# Autodesk Inventor assembly: steelSlides350mm3.0
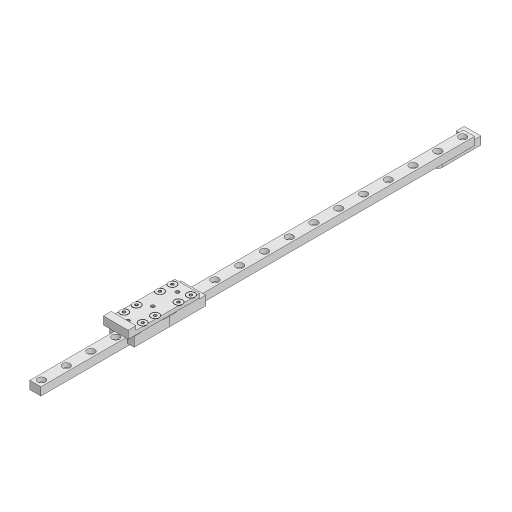
[picture p0: Inventor's stored thumbnail of the model, 512x512]
Saved by Autodesk Inventor 2023 (Build 270158000, 158)
## iProperties
Created: 2022-09-16
Part Number: steelSlides350mm3.0
Document SubType Name: Assembly
Designer: deli
Author: deli
## Documents named in this file (7)
- C:\Users\deli\OneDrive - Eastside Preparatory School\FTC\8103-power-play\CAD\steelSlides350mm3.0.iam
- C:\Users\deli\OneDrive - Eastside Preparatory School\FTC\8103-power-play\CAD\Rail.ipt
- C:\Users\deli\OneDrive - Eastside Preparatory School\FTC\8103-power-play\CAD\Carrige.ipt
- C:\Users\deli\OneDrive - Eastside Preparatory School\FTC\8103-power-play\CAD\Carrige Attatchment.ipt
- C:\Users\deli\OneDrive - Eastside Preparatory School\FTC\8103-power-play\CAD\FTC-parts\Mcmaster Carr\91294A126_Black-Oxide Alloy Steel Hex Drive Flat Head Screw.ipt
- C:\Users\deli\OneDrive - Eastside Preparatory School\FTC\8103-power-play\CAD\mgn9 350mm.ipt
- C:\Users\deli\OneDrive - Eastside Preparatory School\FTC\8103-power-play\CAD\mgn9SlideBearingHolder.ipt
## Components (14 placed, 6 different names)
1. Carrige:3 — Flush:1, Flush:2, Mate:1, Mate:9, Mate:10
2. Carrige:4 — Flush:1, Flush:2, Mate:1, Mate:4, Mate:22, Mate:23
3. Carrige Attatchment:1 — Mate:4, Mate:9, Mate:10, Mate:11, Mate:12, Mate:13, Mate:14, Mate:15, Mate:16, Mate:17, Mate:18, Mate:19, Mate:20, Mate:21, Flush:3, Flush:4, Flush:5, Flush:6, Flush:7, Flush:8, Flush:9, Flush:10
4. Rail:2 — Mate:11, Mate:12, Mate:13
5. 91294A126_Black-Oxide Alloy Steel Hex Drive Flat Head Screw:1 — Mate:20, Flush:8
6. 91294A126_Black-Oxide Alloy Steel Hex Drive Flat Head Screw:2 — Mate:21, Flush:10
7. 91294A126_Black-Oxide Alloy Steel Hex Drive Flat Head Screw:3 — Mate:16, Flush:4
8. 91294A126_Black-Oxide Alloy Steel Hex Drive Flat Head Screw:4 — Mate:15, Flush:3
9. 91294A126_Black-Oxide Alloy Steel Hex Drive Flat Head Screw:5 — Mate:17, Flush:7
10. 91294A126_Black-Oxide Alloy Steel Hex Drive Flat Head Screw:6 — Mate:18, Flush:6
11. 91294A126_Black-Oxide Alloy Steel Hex Drive Flat Head Screw:7 — Mate:19, Flush:9
12. 91294A126_Black-Oxide Alloy Steel Hex Drive Flat Head Screw:8 — Mate:14, Flush:5
13. mgn9 350mm:1 — Mate:22, Mate:23, Mate:24, Mate:25, Mate:26
14. mgn9SlideBearingHolder:1 — Mate:24, Mate:25, Mate:26
## Relationships (30: Mate 20, Flush 10)
- Flush:1: Carrige:3 ↔ Carrige:4
- Flush:2: Carrige:3 ↔ Carrige:4
- Mate:1: Carrige:3 ↔ Carrige:4
- Mate:4: Carrige:4 ↔ Carrige Attatchment:1
- Mate:9: Carrige:3 ↔ Carrige Attatchment:1
- Mate:10: Carrige:3 ↔ Carrige Attatchment:1
- Mate:11: Carrige Attatchment:1 ↔ Rail:2
- Mate:12: Carrige Attatchment:1 ↔ Rail:2
- Mate:13: Carrige Attatchment:1 ↔ Rail:2
- Mate:14: Carrige Attatchment:1 ↔ 91294A126_Black-Oxide Alloy Steel Hex Drive Flat Head Screw:8
- Mate:15: Carrige Attatchment:1 ↔ 91294A126_Black-Oxide Alloy Steel Hex Drive Flat Head Screw:4
- Mate:16: Carrige Attatchment:1 ↔ 91294A126_Black-Oxide Alloy Steel Hex Drive Flat Head Screw:3
- Mate:17: Carrige Attatchment:1 ↔ 91294A126_Black-Oxide Alloy Steel Hex Drive Flat Head Screw:5
- Mate:18: Carrige Attatchment:1 ↔ 91294A126_Black-Oxide Alloy Steel Hex Drive Flat Head Screw:6
- Mate:19: Carrige Attatchment:1 ↔ 91294A126_Black-Oxide Alloy Steel Hex Drive Flat Head Screw:7
- Mate:20: Carrige Attatchment:1 ↔ 91294A126_Black-Oxide Alloy Steel Hex Drive Flat Head Screw:1
- Mate:21: Carrige Attatchment:1 ↔ 91294A126_Black-Oxide Alloy Steel Hex Drive Flat Head Screw:2
- Flush:3: Carrige Attatchment:1 ↔ 91294A126_Black-Oxide Alloy Steel Hex Drive Flat Head Screw:4
- Flush:4: Carrige Attatchment:1 ↔ 91294A126_Black-Oxide Alloy Steel Hex Drive Flat Head Screw:3
- Flush:5: Carrige Attatchment:1 ↔ 91294A126_Black-Oxide Alloy Steel Hex Drive Flat Head Screw:8
- Flush:6: Carrige Attatchment:1 ↔ 91294A126_Black-Oxide Alloy Steel Hex Drive Flat Head Screw:6
- Flush:7: Carrige Attatchment:1 ↔ 91294A126_Black-Oxide Alloy Steel Hex Drive Flat Head Screw:5
- Flush:8: Carrige Attatchment:1 ↔ 91294A126_Black-Oxide Alloy Steel Hex Drive Flat Head Screw:1
- Flush:9: Carrige Attatchment:1 ↔ 91294A126_Black-Oxide Alloy Steel Hex Drive Flat Head Screw:7
- Flush:10: Carrige Attatchment:1 ↔ 91294A126_Black-Oxide Alloy Steel Hex Drive Flat Head Screw:2
- Mate:22: Carrige:4 ↔ mgn9 350mm:1
- Mate:23: Carrige:4 ↔ mgn9 350mm:1
- Mate:24: mgn9 350mm:1 ↔ mgn9SlideBearingHolder:1
- Mate:25: mgn9 350mm:1 ↔ mgn9SlideBearingHolder:1
- Mate:26: mgn9 350mm:1 ↔ mgn9SlideBearingHolder:1
## Named parameters: stroke = 242.2 mm
